# Autodesk Inventor assembly: ciggy
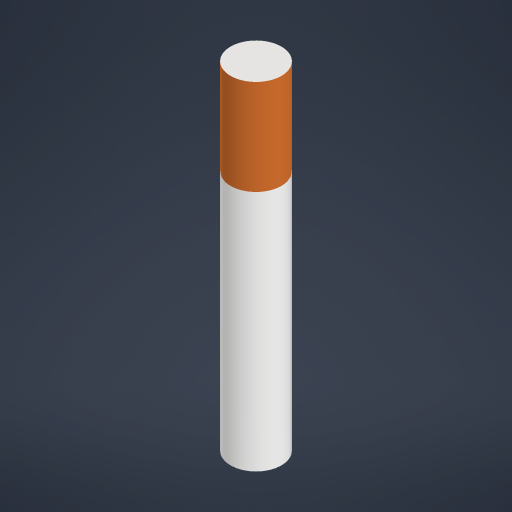
[picture p0: Inventor's stored thumbnail of the model, 512x512]
Saved by Autodesk Inventor 2024 (Build 280153000, 153)
## iProperties
Created: 2025-01-28
Part Number: ciggy
Document SubType Name: Assembly
Designer: turbo
Author: turbo
## Documents named in this file (3)
- C:\Shared\alex-bartella-schoolwork\4b03\ciggy.iam
- C:\Shared\alex-bartella-schoolwork\4b03\ciggy1.ipt
- C:\Shared\alex-bartella-schoolwork\4b03\ciggy2.ipt
## Components (2 placed, 2 different names)
1. ciggy1:1 — Mate:1, Mate:2
2. ciggy2:1 — Mate:1, Mate:2
## Relationships (2: Mate 2)
- Mate:1: ciggy1:1 ↔ ciggy2:1
- Mate:2: ciggy1:1 ↔ ciggy2:1
